# Autodesk Inventor assembly: TorqueLimiter
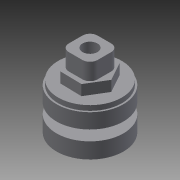
[picture p0: Inventor's stored thumbnail of the model, 180x180]
Saved by Autodesk Inventor 2015 (Build 190159000, 159)
## iProperties
Created: 2015-02-14
Part Number: TorqueLimiter
Document SubType Name: Assembly
Designer: chapale16
Author: chapale16
## Documents named in this file (3)
- \\lhssvr02\Homedirs\Robotics Club\CAD Model 2015\Torque Limiter\TorqueLimiter.iam
- \\lhssvr02\Homedirs\Robotics Club\CAD Model 2015\Torque Limiter\Top.ipt
- \\lhssvr02\Homedirs\Robotics Club\CAD Model 2015\Torque Limiter\Bottom.ipt
## Components (2 placed, 2 different names)
1. Top:1 — Mate:1
2. Bottom:1 — Mate:1
## Relationships (1: Mate 1)
- Mate:1: Top:1 ↔ Bottom:1
